# Autodesk Inventor assembly: ElectricalBoxAssembly
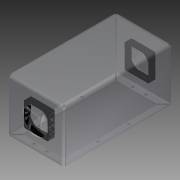
[picture p0: Inventor's stored thumbnail of the model, 180x180]
Saved by Autodesk Inventor 2015 (Build 190159000, 159)
## iProperties
Created: 2015-05-12
Part Number: ElectricalBoxAssembly
Document SubType Name: Assembly
Designer: carpenma
Author: carpenma
## Documents named in this file (3)
- C:\Users\carpe_000\Documents\GitHub\PFPRobot\Mechanical\Drivetrain WIth Cart\Electrical Board-Box\ElectricalBoxAssembly.iam
- C:\Users\carpe_000\Documents\GitHub\PFPRobot\Mechanical\Drivetrain WIth Cart\Electrical Board-Box\60mm Fan Footprint.ipt
- C:\Users\carpe_000\Documents\GitHub\PFPRobot\Mechanical\Drivetrain WIth Cart\Electrical Board-Box\Cover.ipt
## Components (3 placed, 2 different names)
1. 60mm Fan Footprint:1 — Mate:1
2. Cover:1 — Mate:1, Mate:2
3. 60mm Fan Footprint:2 — Mate:2
## Relationships (2: Mate 2)
- Mate:1: 60mm Fan Footprint:1 ↔ Cover:1
- Mate:2: Cover:1 ↔ 60mm Fan Footprint:2
